# Autodesk Inventor assembly: ASY PNS-001 left module
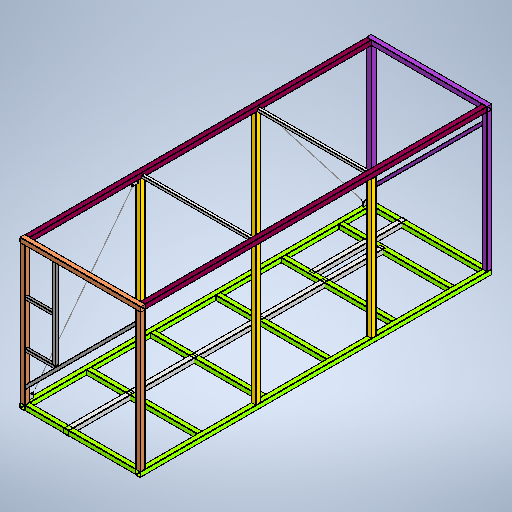
[picture p0: Inventor's stored thumbnail of the model, 512x512]
Saved by Autodesk Inventor 2025 (Build 290162010, 162A)
## iProperties
Created: 2025-03-25
Part Number: ASY PNS-001 left module
Document SubType Name: Assembly
Designer: user
Mass: 1.00117e+06 g
Surface Area: 692723 cm^2
Volume: 127418 cm^3
Density: 7.85736 g/cm^3
Author: user
## Documents named in this file (9)
- C:\Users\admin\YandexDisk-badmisterfox\home pc\Inventor\PNS-Panaevsk\ASY PNS-001 left module.iam
- C:\Users\admin\YandexDisk-badmisterfox\home pc\Inventor\PNS-Panaevsk\ASY PNS-0110 frame left floor.iam
- C:\Users\admin\YandexDisk-badmisterfox\home pc\Inventor\PNS-Panaevsk\ASY PNS-0250 frame featheredge 0260.iam
- C:\Users\admin\YandexDisk-badmisterfox\home pc\Inventor\PNS-Panaevsk\ASY PNS-0250 frame featheredge 0270.iam
- C:\Users\admin\YandexDisk-badmisterfox\home pc\Inventor\PNS-Panaevsk\PNS-0261 Upper beam.ipt
- C:\Users\admin\YandexDisk-badmisterfox\home pc\Inventor\PNS-Panaevsk\PNS-0262 middle pillar.ipt
- C:\Users\admin\YandexDisk-badmisterfox\home pc\Inventor\PNS-Panaevsk\PNS-071 stretch ring.ipt
- C:\Users\admin\YandexDisk-badmisterfox\home pc\Inventor\PNS-Panaevsk\PNS-0310 strench.ipt
- C:\Users\admin\YandexDisk-badmisterfox\home pc\Inventor\PNS-Panaevsk\PNS-0262 cross beam.ipt
## Components (17 placed, 8 different names)
1. ASY PNS-0110 frame left floor:1 [sub-assembly]
2. ASY PNS-0250 frame featheredge 0260:1 [sub-assembly] — Rigid:3, Rigid:4, Rigid:6, Rigid:7, Rigid:10
3. ASY PNS-0250 frame featheredge 0270:1 [sub-assembly] — Rigid:5, Rigid:8, Rigid:12
4. PNS-0261 Upper beam:1 — Rigid:3
5. PNS-0261 Upper beam:2 — Rigid:4
6. PNS-0262 middle pillar:1 — Rigid:5, Rigid:11
7. PNS-0262 middle pillar:2 — Rigid:8, Rigid:13
8. PNS-0262 middle pillar:3 — Rigid:7, Rigid:14
9. PNS-0262 middle pillar:4 — Rigid:6, Rigid:9
10. PNS-071 stretch ring:1 — Rigid:9, Mate:1, Flush:1
11. PNS-071 stretch ring:2 — Rigid:10
12. PNS-0310 strench:1 — Mate:1, Flush:1
13. PNS-071 stretch ring:3 — Rigid:11, Mate:2, Mate:3
14. PNS-071 stretch ring:4 — Rigid:12
15. PNS-0310 strench:2 — Mate:2, Mate:3
16. PNS-0262 cross beam:1 — Rigid:13
17. PNS-0262 cross beam:2 — Rigid:14
## Relationships (18: WeldJoint 14, Mate 3, Flush 1)
- [WeldJoint]: ASY PNS-0110 frame left floor:1 ↔ ASY PNS-0250 frame featheredge 0260:1
- [WeldJoint]: ASY PNS-0110 frame left floor:1 ↔ ASY PNS-0250 frame featheredge 0270:1
- Rigid:3 [WeldJoint]: ASY PNS-0250 frame featheredge 0260:1 ↔ PNS-0261 Upper beam:1
- Rigid:4 [WeldJoint]: ASY PNS-0250 frame featheredge 0260:1 ↔ PNS-0261 Upper beam:2
- Rigid:5 [WeldJoint] (2200 mm): ASY PNS-0250 frame featheredge 0270:1 ↔ PNS-0262 middle pillar:1
- Rigid:6 [WeldJoint] (2200 mm): ASY PNS-0250 frame featheredge 0260:1 ↔ PNS-0262 middle pillar:4
- Rigid:7 [WeldJoint] (2200 mm): ASY PNS-0250 frame featheredge 0260:1 ↔ PNS-0262 middle pillar:3
- Rigid:8 [WeldJoint] (2200 mm): ASY PNS-0250 frame featheredge 0270:1 ↔ PNS-0262 middle pillar:2
- Rigid:9 [WeldJoint]: PNS-0262 middle pillar:4 ↔ PNS-071 stretch ring:1
- Rigid:10 [WeldJoint]: ASY PNS-0250 frame featheredge 0260:1 ↔ PNS-071 stretch ring:2
- Rigid:11 [WeldJoint]: PNS-0262 middle pillar:1 ↔ PNS-071 stretch ring:3
- Rigid:12 [WeldJoint]: ASY PNS-0250 frame featheredge 0270:1 ↔ PNS-071 stretch ring:4
- Mate:1: PNS-071 stretch ring:1 ↔ PNS-0310 strench:1
- Flush:1: PNS-071 stretch ring:1 ↔ PNS-0310 strench:1
- Mate:2: PNS-071 stretch ring:3 ↔ PNS-0310 strench:2
- Mate:3: PNS-071 stretch ring:3 ↔ PNS-0310 strench:2
- Rigid:13 [WeldJoint]: PNS-0262 middle pillar:2 ↔ PNS-0262 cross beam:1
- Rigid:14 [WeldJoint]: PNS-0262 middle pillar:3 ↔ PNS-0262 cross beam:2
